# Autodesk Inventor assembly: ensemble
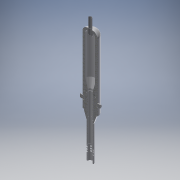
[picture p0: Inventor's stored thumbnail of the model, 180x180]
Saved by Autodesk Inventor 2019 (Build 230136000, 136)
## iProperties
Created: 2018-04-17
Part Number: ensemble
Material: Générique
Document SubType Name: Assembly
Designer: Theo
Author: Theo
## Documents named in this file (6)
- D:\dev\projects\canon-ace\ACE 12 1\ensemble.iam
- D:\dev\projects\canon-ace\ACE 12 1\reservoir.ipt
- D:\dev\projects\canon-ace\ACE 12 1\joint.ipt
- D:\dev\projects\canon-ace\ACE 12 1\canon.ipt
- D:\dev\projects\canon-ace\ACE 12 1\douille.ipt
- D:\dev\3d_parts\legris_3166_06_08\3166_06_08.ipt
## Components (5 placed, 5 different names)
1. reservoir:1 — Placage:1, Affleurement:2, Placage:2, Placage:5, Placage:6
2. joint:1 — Placage:1, Affleurement:1
3. canon:1 — Placage:2, Placage:3, Placage:4
4. douille:1 — Placage:3, Placage:4, Placage:5
5. 3166_06_08:1 — Placage:6
## Relationships (8: Mate 6, Flush 2)
- Placage:1 [Mate]: reservoir:1 ↔ joint:1
- Affleurement:1 [Flush] (-3 mm): joint:1
- Affleurement:2 [Flush]: reservoir:1
- Placage:2 [Mate]: reservoir:1 ↔ canon:1
- Placage:3 [Mate]: canon:1 ↔ douille:1
- Placage:4 [Mate]: canon:1 ↔ douille:1
- Placage:5 [Mate]: reservoir:1 ↔ douille:1
- Placage:6 [Mate]: reservoir:1 ↔ 3166_06_08:1
